# Autodesk Inventor assembly: Assembly3
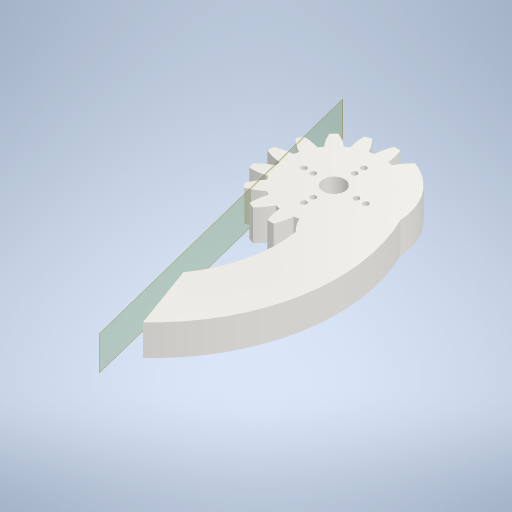
[picture p0: Inventor's stored thumbnail of the model, 512x512]
Saved by Autodesk Inventor 2024 (Build 280153000, 153)
## iProperties
Created: 2023-09-24
Part Number: Assembly3
Document SubType Name: Assembly
Designer: jebes windows
Author: jebes windows
## Documents named in this file (2)
- C:\Users\jebes windows\Documents\Inventor\Robotska_roka\Assembly3.iam
- C:\Users\jebes windows\Documents\Inventor\Robotska_roka\roka_asemb\Design Accelerator\Spur Gear21.ipt
## Components (1 placed, 1 different names)
1. Spur Gear2:1 — Mate:1, Tangent:1
## Relationships (2: Mate 1, Tangent 1)
- Mate:1: Spur Gear2:1
- Tangent:1: Spur Gear2:1
